# Autodesk Inventor assembly: 16 tooth sprocket mount on custom clamping hub
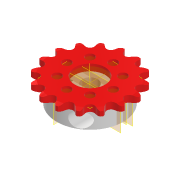
[picture p0: Inventor's stored thumbnail of the model, 180x180]
Saved by Autodesk Inventor 2020 (Build 240168000, 168)
## iProperties
Created: 2020-01-31
Part Number: 16 tooth sprocket mount on custom clamping hub
Document SubType Name: Assembly
Designer: ball
Author: ball
## Documents named in this file (3)
- C:\FTC\FTC8863CAD\2019 Robot\Delivery\extension arm\16 tooth sprocket mount on custom clamping hub.iam
- C:\FTC\FTC8863CAD\2019 Robot\Generic Parts\clamping hub .770 .25 D bore base.ipt
- C:\FTC\FTC8863CAD\Actobotics\615 parts\615102.ipt
## Components (2 placed, 2 different names)
1. clamping hub .770 .25 D bore base:1 — Mate:1, Mate:2, Mate:3
2. 615102:1 — Mate:1, Mate:2, Mate:3
## Relationships (3: Mate 3)
- Mate:1: clamping hub .770 .25 D bore base:1 ↔ 615102:1
- Mate:2: clamping hub .770 .25 D bore base:1 ↔ 615102:1
- Mate:3: clamping hub .770 .25 D bore base:1 ↔ 615102:1
